# Autodesk Inventor assembly: Assembly1
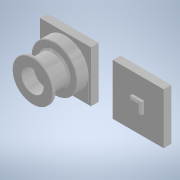
[picture p0: Inventor's stored thumbnail of the model, 180x180]
Saved by Autodesk Inventor 2022 (Build 260153000, 153)
## iProperties
Created: 2022-12-01
Part Number: Assembly1
Document SubType Name: Assembly
Designer: Aiden
Author: Aiden
## Documents named in this file (3)
- C:\Users\Aiden\Documents\KiCAD\Underwater Tactile Sensor\V1\3d models\Assembly1.iam
- C:\Users\Aiden\Documents\KiCAD\Underwater Tactile Sensor\V1\3d models\MS5837-30BA.ipt
- C:\Users\Aiden\Documents\KiCAD\Underwater Tactile Sensor\V1\3d models\MS5837-30BA-exposed-crystal.ipt
## Components (2 placed, 2 different names)
1. MS5837-30BA:1 — Flush:1, Flush:2
2. MS5837-30BA-exposed-crystal:1 — Flush:1, Flush:2
## Relationships (2: Flush 2)
- Flush:1: MS5837-30BA:1 ↔ MS5837-30BA-exposed-crystal:1
- Flush:2: MS5837-30BA:1 ↔ MS5837-30BA-exposed-crystal:1
